# Autodesk Inventor assembly: transmission main
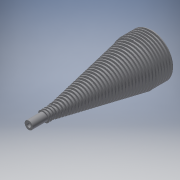
[picture p0: Inventor's stored thumbnail of the model, 180x180]
Saved by Autodesk Inventor 2018 (Build 220112000, 112)
## iProperties
Created: 2018-10-26
Part Number: transmission main
Document SubType Name: Assembly
Designer: 871357
Author: 871357
## Documents named in this file (4)
- L:\POE\transmission main.iam
- L:\POE\TransmissionTorque.ipt
- L:\POE\Transmission2.ipt
- L:\POE\TransmissionTop.ipt
## Components (3 placed, 3 different names)
1. TransmissionTorque:1 — Mate:1
2. Transmission2:1 — Mate:1, Mate:2
3. TransmissionTop:1 — Mate:2
## Relationships (2: Mate 2)
- Mate:1: TransmissionTorque:1 ↔ Transmission2:1
- Mate:2: Transmission2:1 ↔ TransmissionTop:1
